# Autodesk Inventor assembly: board_compelite
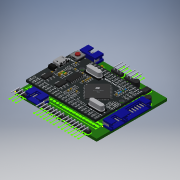
[picture p0: Inventor's stored thumbnail of the model, 180x180]
Saved by Autodesk Inventor 2019 (Build 230136000, 136)
## iProperties
Created: 2020-03-08
Part Number: board_compelite
Document SubType Name: Assembly
Designer: Pulag
Author: Pulag
## Documents named in this file (5)
- C:\Users\Pulag\Desktop\CAD\board_compelite.iam
- C:\Users\Pulag\Desktop\New folder\board.ipt
- C:\Users\Pulag\Desktop\CAD\MEGA 2560 PRO (EMBED).iam
- C:\Users\Pulag\Desktop\CAD\B4B-PH-SM4-TB.ipt
- C:\Users\Pulag\Desktop\CAD\B8B-PH-SM4-TB.ipt
## Components (6 placed, 4 different names)
1. board:1 — Flush:1, Mate:1, Mate:2, Mate:3, Mate:4, Mate:5, Mate:6, Mate:7, Mate:8, Mate:9, Mate:10, Mate:11, Mate:12, Mate:13, Mate:14
2. MEGA 2560 PRO (EMBED):1 [sub-assembly] — Flush:1, Mate:5, Mate:6
3. B4B-PH-SM4-TB:1 — Mate:1, Mate:4, Mate:11
4. B4B-PH-SM4-TB:2 — Mate:2, Mate:7, Mate:10
5. B4B-PH-SM4-TB:3 — Mate:3, Mate:8, Mate:9
6. B8B-PH-SM4-TB:1 — Mate:12, Mate:13, Mate:14
## Relationships (15: Mate 14, Flush 1)
- Flush:1 (-6 mm): board:1 ↔ MEGA 2560 PRO (EMBED):1
- Mate:1: board:1 ↔ B4B-PH-SM4-TB:1
- Mate:2: board:1 ↔ B4B-PH-SM4-TB:2
- Mate:3: board:1 ↔ B4B-PH-SM4-TB:3
- Mate:4: board:1 ↔ B4B-PH-SM4-TB:1
- Mate:5: board:1 ↔ MEGA 2560 PRO (EMBED):1
- Mate:6: board:1 ↔ MEGA 2560 PRO (EMBED):1
- Mate:7: board:1 ↔ B4B-PH-SM4-TB:2
- Mate:8: board:1 ↔ B4B-PH-SM4-TB:3
- Mate:9 (-0.975 mm): board:1 ↔ B4B-PH-SM4-TB:3
- Mate:10 (-0.975 mm): board:1 ↔ B4B-PH-SM4-TB:2
- Mate:11 (-0.975 mm): board:1 ↔ B4B-PH-SM4-TB:1
- Mate:12: board:1 ↔ B8B-PH-SM4-TB:1
- Mate:13: board:1 ↔ B8B-PH-SM4-TB:1
- Mate:14 (-0.975 mm): board:1 ↔ B8B-PH-SM4-TB:1
